# Autodesk Inventor assembly: inner_frame
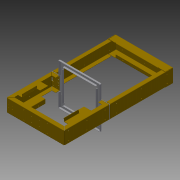
[picture p0: Inventor's stored thumbnail of the model, 180x180]
Saved by Autodesk Inventor 2014 SP2 (Build 180246200, 246)
## iProperties
Created: 2016-05-21
Part Number: inner_frame
Document SubType Name: Assembly
Designer: cruiser
Author: cruiser
## Documents named in this file (4)
- C:\Users\cruiser\Desktop\models\3d printers\laserresin4\inner_frame.iam
- C:\Users\cruiser\Desktop\models\3d printers\laserresin4\carrier.ipt
- C:\Users\cruiser\Desktop\models\3d printers\laserresin4\frame_inner.ipt
- C:\Users\cruiser\Desktop\models\3d printers\laserresin4\frame_lower.ipt
## Components (3 placed, 3 different names)
1. carrier:1 — Mate:1, Mate:2, Mate:3, Mate:4, Mate:5, Mate:6
2. frame_inner:1 — Mate:1, Mate:3, Mate:4
3. frame_lower:1 — Mate:2, Mate:5, Mate:6
## Relationships (6: Mate 6)
- Mate:1: carrier:1 ↔ frame_inner:1
- Mate:2: carrier:1 ↔ frame_lower:1
- Mate:3: carrier:1 ↔ frame_inner:1
- Mate:4: carrier:1 ↔ frame_inner:1
- Mate:5: carrier:1 ↔ frame_lower:1
- Mate:6: carrier:1 ↔ frame_lower:1
